# Autodesk Inventor assembly: Base 2.0
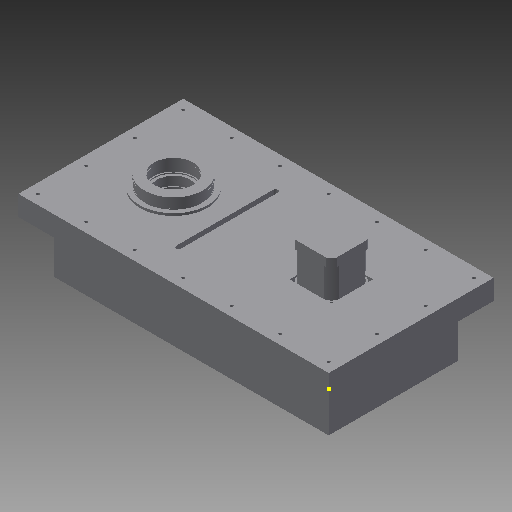
[picture p0: Inventor's stored thumbnail of the model, 512x512]
Saved by Autodesk Inventor 2019 (Build 230136000, 136)
## iProperties
Created: 2021-11-07
Part Number: Base 2.0
Document SubType Name: Assembly
Designer: Mohamed
Author: Mohamed
## Documents named in this file (11)
- D:\mody\IndustrialLine\SortingAndStorage\Inventor\SSCARA Robot\Base 2.0.iam
- D:\mody\IndustrialLine\SortingAndStorage\Inventor\SSCARA Robot\b_base_support 3.ipt
- D:\mody\IndustrialLine\SortingAndStorage\Inventor\SSCARA Robot\b_base_support 2.ipt
- D:\mody\IndustrialLine\SortingAndStorage\Inventor\SSCARA Robot\b_Base_support 1.ipt
- D:\mody\IndustrialLine\SortingAndStorage\Inventor\SSCARA Robot\thrust bearing_40mm.iam
- D:\mody\IndustrialLine\SortingAndStorage\Inventor\SSCARA Robot\b_base_cover_1.ipt
- D:\mody\IndustrialLine\SortingAndStorage\Inventor\SSCARA Robot\nema 17 motor.ipt
- D:\mody\IndustrialLine\SortingAndStorage\Inventor\SSCARA Robot\ball bearing 35mm.ipt
- D:\mody\IndustrialLine\SortingAndStorage\Inventor\SSCARA Robot\GT2 pulley 20 teeth.ipt
- D:\mody\IndustrialLine\SortingAndStorage\Inventor\SSCARA Robot\belt_460mm.ipt
- D:\mody\IndustrialLine\SortingAndStorage\Inventor\SSCARA Robot\B_thrust bearing _support.ipt
## Components (13 placed, 10 different names)
1. b_base_support 3:1 — Mate:4, Flush:1, Flush:2
2. b_base_support 2:1 — Mate:6, Flush:5, Flush:6
3. b_Base_support 1:1 — Mate:1, Mate:2, Mate:3, Mate:4, Flush:1, Mate:5, Flush:3, Mate:6, Flush:6, Mate:19, Flush:8, Flush:9
4. b_base_support 3:2 — Mate:5, Flush:3, Flush:4, Flush:5
5. b_base_support 2:2 — Mate:1, Mate:2, Mate:3, Flush:2, Flush:4
6. thrust bearing_40mm:1 [sub-assembly] — Mate:12
7. thrust bearing_40mm:2 [sub-assembly] — Mate:13, Mate:25
8. b_base_cover_1:1 — Mate:9, Mate:10, Mate:12, Mate:13, Mate:15, Mate:16, Mate:17, Mate:19, Flush:8, Flush:9, Mate:26
9. nema 17 motor:1 — Mate:15, Mate:16, Mate:17, Mate:18
10. ball bearing 35mm:1 — Mate:9, Mate:10
11. GT2 pulley 20 teeth:1 — Mate:18, Mate:20, Mate:22
12. belt_460mm:1 — Mate:20, Mate:22
13. B_thrust bearing _support:1 — Mate:25, Mate:26
## Relationships (27: Mate 19, Flush 8)
- Mate:1: b_Base_support 1:1 ↔ b_base_support 2:2
- Mate:2: b_Base_support 1:1 ↔ b_base_support 2:2
- Mate:3: b_Base_support 1:1 ↔ b_base_support 2:2
- Mate:4: b_base_support 3:1 ↔ b_Base_support 1:1
- Flush:1: b_base_support 3:1 ↔ b_Base_support 1:1
- Flush:2: b_base_support 3:1 ↔ b_base_support 2:2
- Mate:5: b_Base_support 1:1 ↔ b_base_support 3:2
- Flush:3: b_Base_support 1:1 ↔ b_base_support 3:2
- Flush:4: b_base_support 3:2 ↔ b_base_support 2:2
- Mate:6: b_base_support 2:1 ↔ b_Base_support 1:1
- Flush:5: b_base_support 2:1 ↔ b_base_support 3:2
- Flush:6: b_base_support 2:1 ↔ b_Base_support 1:1
- Mate:9: b_base_cover_1:1 ↔ ball bearing 35mm:1
- Mate:10: b_base_cover_1:1 ↔ ball bearing 35mm:1
- Mate:12: thrust bearing_40mm:1 ↔ b_base_cover_1:1
- Mate:13: thrust bearing_40mm:2 ↔ b_base_cover_1:1
- Mate:15: b_base_cover_1:1 ↔ nema 17 motor:1
- Mate:16: b_base_cover_1:1 ↔ nema 17 motor:1
- Mate:17: b_base_cover_1:1 ↔ nema 17 motor:1
- Mate:18: nema 17 motor:1 ↔ GT2 pulley 20 teeth:1
- Mate:19: b_Base_support 1:1 ↔ b_base_cover_1:1
- Flush:8: b_Base_support 1:1 ↔ b_base_cover_1:1
- Flush:9: b_Base_support 1:1 ↔ b_base_cover_1:1
- Mate:20: GT2 pulley 20 teeth:1 ↔ belt_460mm:1
- Mate:22: GT2 pulley 20 teeth:1 ↔ belt_460mm:1
- Mate:25: thrust bearing_40mm:2 ↔ B_thrust bearing _support:1
- Mate:26: b_base_cover_1:1 ↔ B_thrust bearing _support:1
